# Autodesk Inventor assembly: Frame
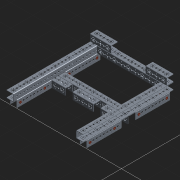
[picture p0: Inventor's stored thumbnail of the model, 180x180]
Saved by Autodesk Inventor 2015 SP1 (Build 190203100, 203)
## iProperties
Created: 2015-01-22
Part Number: Frame
Document SubType Name: Assembly
Designer: rihoobler
Author: rihoobler
## Documents named in this file (6)
- C:\Users\datenney\Documents\GitHub\CAD\SerenityMk.2\Frame.iam
- C:\Users\datenney\Documents\GitHub\CAD\SerenityMk.2\Frame Long Side.iam
- C:\Users\datenney\Documents\GitHub\CAD\SerenityMk.2\Imported Components\tetrix_739067_2012_160_channel\tetrix_739067_2012_160_channel.ipt
- C:\Users\datenney\Documents\GitHub\CAD\SerenityMk.2\Imported Components\tetrix_739068_2012_288_channel\tetrix_739068_2012_288_channel.ipt
- C:\Users\datenney\Documents\GitHub\CAD\SerenityMk.2\Imported Components\tetrix_739066_2012_96_channel\tetrix_739066_2012_96_channel.ipt
- C:\Users\datenney\Documents\GitHub\CAD\SerenityMk.2\Imported Components\tetrix_739091_2012\tetrix_739091_2012.ipt
## Components (29 placed, 5 different names)
1. Frame Long Side:1 [sub-assembly] — Flush:1, Flush:2, Flush:5, Mate:5, Mate:6, Flush:6, Mate:7, Mate:8, Mate:16, Flush:13, Mate:21, Mate:22
2. Frame Long Side:2 [sub-assembly] — Flush:1, Flush:2, Mate:1, Flush:3, Mate:2, Flush:4, Mate:3, Mate:4, Mate:15, Mate:17
3. tetrix_739067_2012_160_channel:1 — Mate:1, Flush:3, Mate:2, Insert:3, Insert:6, Insert:13, Insert:14
4. tetrix_739067_2012_160_channel:2 — Flush:4, Mate:3, Mate:4, Insert:2, Insert:5, Insert:11, Insert:12
5. tetrix_739067_2012_160_channel:3 — Flush:6, Mate:7, Mate:8, Insert:9, Insert:10, Insert:15, Insert:16
6. tetrix_739067_2012_160_channel:4 — Flush:5, Mate:5, Mate:6, Insert:7, Insert:8, Insert:17, Insert:18
7. tetrix_739068_2012_288_channel:1 — Mate:9, Flush:7, Mate:10, Mate:11, Flush:8, Mate:12, Mate:13, Flush:9, Mate:14
8. tetrix_739066_2012_96_channel:1 — Mate:9, Flush:7, Mate:10, Mate:17
9. tetrix_739066_2012_96_channel:2 — Mate:11, Flush:8, Mate:12, Mate:15, Mate:16
10. tetrix_739066_2012_96_channel:3 — Mate:13, Flush:9, Mate:14
11. tetrix_739091_2012:1 — Insert:5
12. tetrix_739091_2012:2 — Insert:2
13. tetrix_739091_2012:3 — Insert:3
14. tetrix_739091_2012:4 — Insert:6
15. tetrix_739091_2012:5 — Insert:11
16. tetrix_739091_2012:6 — Insert:14
17. tetrix_739091_2012:7 — Insert:12
18. tetrix_739091_2012:8 — Insert:13
19. tetrix_739091_2012:9 — Insert:7
20. tetrix_739091_2012:10 — Insert:9
21. tetrix_739091_2012:11 — Insert:8
22. tetrix_739091_2012:12 — Insert:10
23. tetrix_739091_2012:13 — Insert:15
24. tetrix_739091_2012:14 — Insert:16
25. tetrix_739091_2012:15 — Insert:17
26. tetrix_739091_2012:16 — Insert:18
27. tetrix_739068_2012_288_channel:2 — Mate:18, Mate:19, Mate:20, Flush:11
28. tetrix_739066_2012_96_channel:4 — Mate:19, Mate:20, Flush:10, Flush:12
29. tetrix_739066_2012_96_channel:5 — Mate:18, Flush:10, Flush:11, Flush:12, Flush:13, Mate:21, Mate:22
## Relationships (51: Mate 22, Insert 16, Flush 13)
- Flush:1: Frame Long Side:1 ↔ Frame Long Side:2
- Flush:2: Frame Long Side:1 ↔ Frame Long Side:2
- Mate:1: Frame Long Side:2 ↔ tetrix_739067_2012_160_channel:1
- Flush:3: Frame Long Side:2 ↔ tetrix_739067_2012_160_channel:1
- Mate:2: Frame Long Side:2 ↔ tetrix_739067_2012_160_channel:1
- Flush:4: Frame Long Side:2 ↔ tetrix_739067_2012_160_channel:2
- Mate:3: Frame Long Side:2 ↔ tetrix_739067_2012_160_channel:2
- Mate:4: Frame Long Side:2 ↔ tetrix_739067_2012_160_channel:2
- Flush:5: Frame Long Side:1 ↔ tetrix_739067_2012_160_channel:4
- Mate:5: Frame Long Side:1 ↔ tetrix_739067_2012_160_channel:4
- Mate:6: Frame Long Side:1 ↔ tetrix_739067_2012_160_channel:4
- Flush:6: Frame Long Side:1 ↔ tetrix_739067_2012_160_channel:3
- Mate:7: Frame Long Side:1 ↔ tetrix_739067_2012_160_channel:3
- Mate:8: Frame Long Side:1 ↔ tetrix_739067_2012_160_channel:3
- Mate:9: tetrix_739068_2012_288_channel:1 ↔ tetrix_739066_2012_96_channel:1
- Flush:7: tetrix_739068_2012_288_channel:1 ↔ tetrix_739066_2012_96_channel:1
- Mate:10: tetrix_739068_2012_288_channel:1 ↔ tetrix_739066_2012_96_channel:1
- Mate:11: tetrix_739068_2012_288_channel:1 ↔ tetrix_739066_2012_96_channel:2
- Flush:8: tetrix_739068_2012_288_channel:1 ↔ tetrix_739066_2012_96_channel:2
- Mate:12: tetrix_739068_2012_288_channel:1 ↔ tetrix_739066_2012_96_channel:2
- Mate:13: tetrix_739068_2012_288_channel:1 ↔ tetrix_739066_2012_96_channel:3
- Flush:9: tetrix_739068_2012_288_channel:1 ↔ tetrix_739066_2012_96_channel:3
- Mate:14: tetrix_739068_2012_288_channel:1 ↔ tetrix_739066_2012_96_channel:3
- Mate:15: Frame Long Side:2 ↔ tetrix_739066_2012_96_channel:2
- Mate:16: Frame Long Side:1 ↔ tetrix_739066_2012_96_channel:2
- Mate:17: Frame Long Side:2 ↔ tetrix_739066_2012_96_channel:1
- Insert:2: tetrix_739067_2012_160_channel:2 ↔ tetrix_739091_2012:2
- Insert:3: tetrix_739067_2012_160_channel:1 ↔ tetrix_739091_2012:3
- Insert:5: tetrix_739067_2012_160_channel:2 ↔ tetrix_739091_2012:1
- Insert:6: tetrix_739067_2012_160_channel:1 ↔ tetrix_739091_2012:4
- Insert:7: tetrix_739067_2012_160_channel:4 ↔ tetrix_739091_2012:9
- Insert:8: tetrix_739067_2012_160_channel:4 ↔ tetrix_739091_2012:11
- Insert:9: tetrix_739067_2012_160_channel:3 ↔ tetrix_739091_2012:10
- Insert:10: tetrix_739067_2012_160_channel:3 ↔ tetrix_739091_2012:12
- Insert:11: tetrix_739067_2012_160_channel:2 ↔ tetrix_739091_2012:5
- Insert:12: tetrix_739067_2012_160_channel:2 ↔ tetrix_739091_2012:7
- Insert:13: tetrix_739067_2012_160_channel:1 ↔ tetrix_739091_2012:8
- Insert:14: tetrix_739067_2012_160_channel:1 ↔ tetrix_739091_2012:6
- Insert:15: tetrix_739067_2012_160_channel:3 ↔ tetrix_739091_2012:13
- Insert:16: tetrix_739067_2012_160_channel:3 ↔ tetrix_739091_2012:14
- Insert:17: tetrix_739067_2012_160_channel:4 ↔ tetrix_739091_2012:15
- Insert:18: tetrix_739067_2012_160_channel:4 ↔ tetrix_739091_2012:16
- Mate:18: tetrix_739068_2012_288_channel:2 ↔ tetrix_739066_2012_96_channel:5
- Mate:19: tetrix_739068_2012_288_channel:2 ↔ tetrix_739066_2012_96_channel:4
- Mate:20: tetrix_739068_2012_288_channel:2 ↔ tetrix_739066_2012_96_channel:4
- Flush:10: tetrix_739066_2012_96_channel:4 ↔ tetrix_739066_2012_96_channel:5
- Flush:11: tetrix_739068_2012_288_channel:2 ↔ tetrix_739066_2012_96_channel:5
- Flush:12: tetrix_739066_2012_96_channel:4 ↔ tetrix_739066_2012_96_channel:5
- Flush:13: Frame Long Side:1 ↔ tetrix_739066_2012_96_channel:5
- Mate:21: Frame Long Side:1 ↔ tetrix_739066_2012_96_channel:5
- Mate:22: Frame Long Side:1 ↔ tetrix_739066_2012_96_channel:5
